# Autodesk Inventor assembly: 2AM-17-A-0200 - slider motor and gearbox
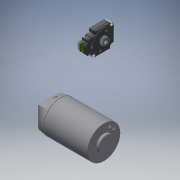
[picture p0: Inventor's stored thumbnail of the model, 180x180]
Saved by Autodesk Inventor 2017 (Build 210142000, 142)
## iProperties
Created: 2017-12-28
Part Number: 2AM-17-A-0200 - slider motor and gearbox
Document SubType Name: Assembly
Designer: Micah
Author: Micah
## Documents named in this file (4)
- C:\Users\Micah\Desktop\inventor\CADathon-2017\2AM-17-A-0200 - Smokestack Elevator\2AM-17-A-0200 - slider motor and gearbox.iam
- C:\Users\Micah\Desktop\inventor\COTS\Motors\Mini CIM Motor\217-3371-STEP.ipt
- C:\Users\Micah\Desktop\inventor\CADathon-2017\2AM-17-A-0200 - Smokestack Elevator\COTS\VersaPlanetary_Integrated_Encoder_217-5046.iam
- C:\Users\Micah\Desktop\inventor\CADathon-2017\2AM-17-A-0200 - Smokestack Elevator\COTS\VersaPlanetary_CIM_Adapter_217-4018.ipt
## Components (3 placed, 3 different names)
1. 217-3371-STEP:1 — Mate:1
2. VersaPlanetary_Integrated_Encoder_217-5046:1 [sub-assembly]
3. VersaPlanetary_CIM_Adapter_217-4018:1 — Mate:1
## Relationships (1: Mate 1)
- Mate:1: 217-3371-STEP:1 ↔ VersaPlanetary_CIM_Adapter_217-4018:1
